# Autodesk Inventor assembly: J007802
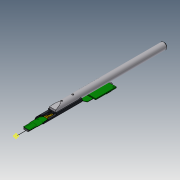
[picture p0: Inventor's stored thumbnail of the model, 180x180]
Saved by Autodesk Inventor 2018.3 (Build 223284000, 284)
## iProperties
Created: 2017-08-07
Vendor: HHMI: JRC - ID&F
Document SubType Name: Assembly
Designer: ARNOLDJ
Project: COMMON
Description: NEUROPIXEL 3A PROBE AND ROD HOLDER
Part Number: J007802
RuleStatus: InUse
AfterDocSave0: file://Part Number Cleaner
DESIGN DEPARTMENT: HHMI: JRC - ID&F
LAB/DEPT: COMMON
REQUESTING SCIENTIST: COMMON
SPECIAL FINISH: N/A
ALTERED ITEM PART NUMBER: N/A
ALTERED ITEM VENDOR: N/A
ALTERED ITEM DESCRIPTION: N/A
Author: ARNOLDJ
Revision Number: 0
## Documents named in this file (7)
- C:\_WORKSPACE\DATA\PROJECTS\_PROJECTS BY LAB\SVOBODA (LAB)\MANIPULATOR FRAME FOR EPHYS\NEUROPIXEL 3A PROBE AND ROD HOLDER.iam
- C:\_WORKSPACE\DATA\PROJECTS\_PROJECTS BY LAB\SVOBODA (LAB)\MANIPULATOR FRAME FOR EPHYS\CUSTOM PARTS\PTR PROBE MOUNT ROD EXTENDED.ipt
- C:\_WORKSPACE\DATA\COMMON\McMaster\92010A003_METRIC 18-8 SS FLAT HEAD PHIL MACHINE SCREW.ipt
- C:\_WORKSPACE\DATA\PROJECTS\_PROJECTS BY LAB\SVOBODA (LAB)\MANIPULATOR FRAME FOR EPHYS\PURCHASED PARTS\NEUROPIXEL 3A PROBE.ipt
- C:\_WORKSPACE\DATA\PROJECTS\_PROJECTS BY LAB\SVOBODA (LAB)\MANIPULATOR FRAME FOR EPHYS\PURCHASED PARTS\NEUROPIXEL HEADSTAGE PCB.ipt
- C:\_WORKSPACE\DATA\COMMON\HENKEL\HENKEL 1365868.ipt
- C:\_WORKSPACE\DATA\PROJECTS\_PROJECTS BY LAB\SVOBODA (LAB)\MANIPULATOR FRAME FOR EPHYS\CUSTOM PARTS\NEUROPIXEL 3A PROBE BASE.ipt
## Components (7 placed, 6 different names)
1. NEUROPIXEL HEADSTAGE PCB:1 — Mate:9, Mate:10, Mate:11
2. NEUROPIXEL 3A PROBE:1 — Flush:4, Flush:5, Mate:7, Mate:8, Mate:9, Mate:11, Mate:13
3. NEUROPIXEL 3A PROBE BASE:1 — Flush:5, Mate:5, Mate:7, Angle:1, Mate:12, Flush:6, Mate:14, Flush:7, Mate:15
4. PTR PROBE MOUNT ROD EXTENDED:1 — Mate:5, Mate:12
5. 92010A003_METRIC 18-8 SS FLAT HEAD PHIL MACHINE SCREW:1 — Flush:6, Mate:14
6. 92010A003_METRIC 18-8 SS FLAT HEAD PHIL MACHINE SCREW:2 — Flush:7, Mate:15
7. HENKEL 1365868:1
## Relationships (15: Mate 10, Flush 4, Angle 1)
- Flush:4 (-89.3064 mm): NEUROPIXEL 3A PROBE:1
- Flush:5 (12.7254 mm): NEUROPIXEL 3A PROBE:1 ↔ NEUROPIXEL 3A PROBE BASE:1
- Mate:5: NEUROPIXEL 3A PROBE BASE:1 ↔ PTR PROBE MOUNT ROD EXTENDED:1
- Mate:7: NEUROPIXEL 3A PROBE:1 ↔ NEUROPIXEL 3A PROBE BASE:1
- Angle:1 (0 deg): NEUROPIXEL 3A PROBE BASE:1
- Mate:8: NEUROPIXEL 3A PROBE:1
- Mate:9: NEUROPIXEL HEADSTAGE PCB:1 ↔ NEUROPIXEL 3A PROBE:1
- Mate:10: NEUROPIXEL HEADSTAGE PCB:1
- Mate:11: NEUROPIXEL HEADSTAGE PCB:1 ↔ NEUROPIXEL 3A PROBE:1
- Mate:12: NEUROPIXEL 3A PROBE BASE:1 ↔ PTR PROBE MOUNT ROD EXTENDED:1
- Mate:13: NEUROPIXEL 3A PROBE:1
- Flush:6 (0.254 mm): NEUROPIXEL 3A PROBE BASE:1 ↔ 92010A003_METRIC 18-8 SS FLAT HEAD PHIL MACHINE SCREW:1
- Mate:14: NEUROPIXEL 3A PROBE BASE:1 ↔ 92010A003_METRIC 18-8 SS FLAT HEAD PHIL MACHINE SCREW:1
- Flush:7 (0.254 mm): NEUROPIXEL 3A PROBE BASE:1 ↔ 92010A003_METRIC 18-8 SS FLAT HEAD PHIL MACHINE SCREW:2
- Mate:15: NEUROPIXEL 3A PROBE BASE:1 ↔ 92010A003_METRIC 18-8 SS FLAT HEAD PHIL MACHINE SCREW:2
